# Autodesk Inventor assembly: Rev Xrail Assembly
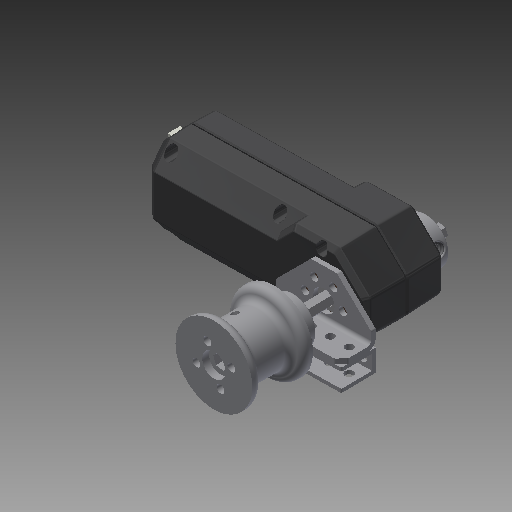
[picture p0: Inventor's stored thumbnail of the model, 512x512]
Saved by Autodesk Inventor 2019 (Build 230136000, 136)
## iProperties
Created: 2019-02-05
Part Number: Rev Xrail Assembly
Document SubType Name: Assembly
Designer: mrhftc
Author: mrhftc
## Documents named in this file (7)
- C:\Users\mrhftc\repositories\design\inventor\Imported Components\REV\Rev Xrail Assembly.iam
- C:\Users\mrhftc\repositories\design\inventor\Imported Components\REV\Motors and Servos\REVCoreHexMotor.ipt
- C:\Users\mrhftc\repositories\design\inventor\Imported Components\REV\Motors and Servos\RevCoreHexMotorMount.ipt
- C:\Users\mrhftc\repositories\design\inventor\Imported Components\REV\Hex Shafts\5mmx75mm_Hex_Shaft.ipt
- C:\Users\mrhftc\repositories\design\inventor\Imported Components\ActoBotics\Mini channel 5 holes\Mini Channel 5 Holes.ipt
- C:\Users\mrhftc\repositories\design\inventor\Imported Components\goBilda\Collar6mm\SetScrewCollar6mmboreassembly.iam
- C:\Users\mrhftc\repositories\design\inventor\2018-2019\Collector Rendition 2.0\Pulley.ipt
## Components (7 placed, 6 different names)
1. REVCoreHexMotor:1 — Rotational:1, Rotational:4, Rotational:5
2. RevCoreHexMotorMount:1 — Rotational:1, Rotational:2
3. 5mmx75mm_Hex_Shaft:1 — Rotational:5
4. Mini Channel 5 Holes:1 — Rotational:2
5. SetScrewCollar6mmboreassembly:1 [sub-assembly] — Rotational:4
6. SetScrewCollar6mmboreassembly:2 [sub-assembly]
7. Pulley:1
## Relationships (4: RevoluteJoint 4)
- Rotational:1 [RevoluteJoint]: REVCoreHexMotor:1 ↔ RevCoreHexMotorMount:1
- Rotational:2 [RevoluteJoint]: RevCoreHexMotorMount:1 ↔ Mini Channel 5 Holes:1
- Rotational:4 [RevoluteJoint]: REVCoreHexMotor:1 ↔ SetScrewCollar6mmboreassembly:1
- Rotational:5 [RevoluteJoint]: REVCoreHexMotor:1 ↔ 5mmx75mm_Hex_Shaft:1
